# Autodesk Inventor assembly: zloz_2
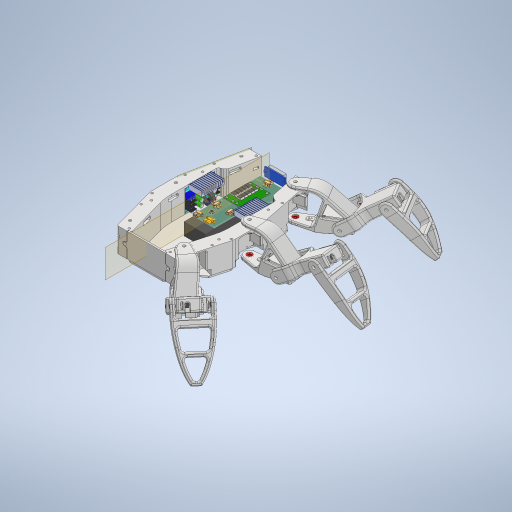
[picture p0: Inventor's stored thumbnail of the model, 512x512]
Saved by Autodesk Inventor 2023.4 (Build 274418000, 418)
## iProperties
Created: 2024-07-26
Part Number: zloz_2
Document SubType Name: Assembly
Designer: kamil
Author: kamil
## Documents named in this file (12)
- E:\PROJECTS_REPOS\Robal-2.0\mechanics\zloz_2.iam
- E:\PROJECTS_REPOS\Robal-2.0\mechanics\Sub-Assy Buck Converter.ipt
- E:\PROJECTS_REPOS\Robal-2.0\mechanics\li_pol_3S_5000mAh.ipt
- E:\PROJECTS_REPOS\Robal-2.0\mechanics\uchwyt_serwa_podwojny.ipt
- E:\PROJECTS_REPOS\Robal-2.0\mechanics\uchwyt_serwa_podwojny_MIR.ipt
- E:\PROJECTS_REPOS\Robal-2.0\mechanics\dol.ipt
- E:\PROJECTS_REPOS\Robal-2.0\mechanics\gora.ipt
- E:\PROJECTS_REPOS\Robal-2.0\mechanics\Lithium Battery Capacity Indicator Module.ipt
- E:\PROJECTS_REPOS\Robal-2.0\mechanics\robal_power_board_2.ipt
- E:\PROJECTS_REPOS\Robal-2.0\mechanics\pokrywa_tyl.ipt
- E:\PROJECTS_REPOS\Robal-2.0\mechanics\pokrywa_przod.ipt
- E:\PROJECTS_REPOS\Robal-2.0\mechanics\noga_pre.iam
## Components (14 placed, 11 different names)
1. Sub-Assy Buck Converter:1 — Równoległe:11, Zestawiające:7, Równoległe:13, Mate:23, Mate:24
2. li_pol_3S_5000mAh:1 — Równoległe:12, Zestawiające:8, Zestawiające:9, Zestawiające:10, Zestawiające:11
3. uchwyt_serwa_podwojny:1 — Równoległe:3, Równoległe:4, Zestawiające:2, Równoległe:9, Symetria:1, Mate:23, Mate:24, Flush:16
4. uchwyt_serwa_podwojny_MIR:1 — Zestawiające:3, Równoległe:5, Równoległe:6, Zestawiające:4, Równoległe:14, Mate:25
5. dol:1 — Zestawiające:1, Równoległe:1, Równoległe:2, Równoległe:3, Równoległe:4, Zestawiające:2, Zestawiające:3, Równoległe:5, Równoległe:6, Równoległe:7, Kątowe:1, Symetria:1, Zestawiające:7, Zestawiające:11, Zestawiające:14, Mate:27
6. gora:1 — Równoległe:1, Równoległe:2, Zestawiające:4, Równoległe:8, Zestawiające:16, Zestawiające:17, Zestawiające:18, Zestawiające:19, Zestawiające:20, Zestawiające:21
7. Lithium Battery Capacity Indicator Module:1 — Równoległe:9, Kątowe:1
8. Sub-Assy Buck Converter:2 — Równoległe:11, Równoległe:13, Mate:25
9. robal_power_board_2:1 — Równoległe:12, Zestawiające:8, Zestawiające:9
10. pokrywa_tyl:1 — Równoległe:14, Zestawiające:14, Równoległe:15
11. pokrywa_przod:1 — Mate:26, Mate:27, Flush:16
12. noga_pre:1 [sub-assembly] — Zestawiające:16, Zestawiające:17
13. noga_pre:2 [sub-assembly] — Zestawiające:18, Zestawiające:20
14. noga_pre:3 [sub-assembly] — Zestawiające:19, Zestawiające:21
## Relationships (38: Mate 21, Flush 15, Angle 1, Symmetry 1)
- Zestawiające:1 [Mate]: dol:1
- Równoległe:1 [Flush]: dol:1 ↔ gora:1
- Równoległe:2 [Flush]: dol:1 ↔ gora:1
- Równoległe:3 [Flush]: uchwyt_serwa_podwojny:1 ↔ dol:1
- Równoległe:4 [Flush]: uchwyt_serwa_podwojny:1 ↔ dol:1
- Zestawiające:2 [Mate]: uchwyt_serwa_podwojny:1 ↔ dol:1
- Zestawiające:3 [Mate]: uchwyt_serwa_podwojny_MIR:1 ↔ dol:1
- Równoległe:5 [Flush]: uchwyt_serwa_podwojny_MIR:1 ↔ dol:1
- Równoległe:6 [Flush]: uchwyt_serwa_podwojny_MIR:1 ↔ dol:1
- Zestawiające:4 [Mate]: uchwyt_serwa_podwojny_MIR:1 ↔ gora:1
- Równoległe:7 [Flush]: dol:1
- Równoległe:8 [Flush]: gora:1
- Równoległe:9 [Flush]: uchwyt_serwa_podwojny:1 ↔ Lithium Battery Capacity Indicator Module:1
- Kątowe:1 [Angle] (0 deg): dol:1 ↔ Lithium Battery Capacity Indicator Module:1
- Symetria:1 [Symmetry]: uchwyt_serwa_podwojny:1 ↔ dol:1
- Równoległe:11 [Flush]: Sub-Assy Buck Converter:1 ↔ Sub-Assy Buck Converter:2
- Zestawiające:7 [Mate]: Sub-Assy Buck Converter:1 ↔ dol:1
- Równoległe:12 [Flush]: li_pol_3S_5000mAh:1 ↔ robal_power_board_2:1
- Zestawiające:8 [Mate]: li_pol_3S_5000mAh:1 ↔ robal_power_board_2:1
- Zestawiające:9 [Mate] (2 mm): li_pol_3S_5000mAh:1 ↔ robal_power_board_2:1
- Zestawiające:10 [Mate] (-22 mm): li_pol_3S_5000mAh:1
- Zestawiające:11 [Mate]: li_pol_3S_5000mAh:1 ↔ dol:1
- Równoległe:13 [Flush]: Sub-Assy Buck Converter:1 ↔ Sub-Assy Buck Converter:2
- Równoległe:14 [Flush]: uchwyt_serwa_podwojny_MIR:1 ↔ pokrywa_tyl:1
- Zestawiające:14 [Mate]: dol:1 ↔ pokrywa_tyl:1
- Równoległe:15 [Flush] (50 mm): pokrywa_tyl:1
- Zestawiające:16 [Mate]: gora:1 ↔ noga_pre:1
- Zestawiające:17 [Mate]: gora:1 ↔ noga_pre:1
- Zestawiające:18 [Mate]: gora:1 ↔ noga_pre:2
- Zestawiające:19 [Mate]: gora:1 ↔ noga_pre:3
- Zestawiające:20 [Mate]: gora:1 ↔ noga_pre:2
- Zestawiające:21 [Mate]: gora:1 ↔ noga_pre:3
- Mate:23: Sub-Assy Buck Converter:1 ↔ uchwyt_serwa_podwojny:1
- Mate:24: Sub-Assy Buck Converter:1 ↔ uchwyt_serwa_podwojny:1
- Mate:25: uchwyt_serwa_podwojny_MIR:1 ↔ Sub-Assy Buck Converter:2
- Mate:26 (-39.25 mm): pokrywa_przod:1
- Mate:27: dol:1 ↔ pokrywa_przod:1
- Flush:16: uchwyt_serwa_podwojny:1 ↔ pokrywa_przod:1
